# Autodesk Inventor assembly: Test Assembly
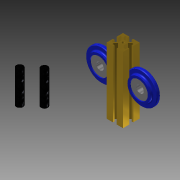
[picture p0: Inventor's stored thumbnail of the model, 180x180]
Saved by Autodesk Inventor 2014 (Build 180170000, 170)
## iProperties
Created: 2015-02-07
Part Number: Test Assembly
Document SubType Name: Assembly
Designer: Spooner
Author: Spooner
## Documents named in this file (5)
- C:\Users\Spooner\Documents\Inventor\80-20  Linear Bearing\Test Assembly.iam
- C:\Users\Spooner\Documents\Inventor\80-20  Linear Bearing\1_5 80-20 x 6in.ipt
- C:\Users\Spooner\Documents\Inventor\80-20  Linear Bearing\Big Bearing.ipt
- C:\Users\Spooner\Documents\Inventor\80-20  Linear Bearing\Big Bearing Cover.ipt
- C:\Users\Spooner\Documents\Inventor\80-20  Linear Bearing\Igus Rod.ipt
## Components (9 placed, 4 different names)
1. 1_5 80-20 x 6in:1 — Mate:1, Mate:2, Mate:6, Flush:2
2. Big Bearing:2 — Mate:1, Flush:2, Insert:1
3. Big Bearing:3 — Mate:2, Mate:6, Insert:2
4. Big Bearing Cover:2 — Insert:1, Insert:3
5. Big Bearing Cover:3 — Insert:2, Insert:5
6. Big Bearing Cover:4 — Insert:5
7. Big Bearing Cover:6 — Insert:3
8. Igus Rod:1
9. Igus Rod:2
## Relationships (8: Insert 4, Mate 3, Flush 1)
- Mate:1: 1_5 80-20 x 6in:1 ↔ Big Bearing:2
- Mate:2: 1_5 80-20 x 6in:1 ↔ Big Bearing:3
- Mate:6 (27.305 mm): 1_5 80-20 x 6in:1 ↔ Big Bearing:3
- Flush:2 (-27.305 mm): 1_5 80-20 x 6in:1 ↔ Big Bearing:2
- Insert:1: Big Bearing:2 ↔ Big Bearing Cover:2
- Insert:2: Big Bearing:3 ↔ Big Bearing Cover:3
- Insert:3: Big Bearing Cover:2 ↔ Big Bearing Cover:6
- Insert:5: Big Bearing Cover:3 ↔ Big Bearing Cover:4
